# Autodesk Inventor assembly: Assembly2
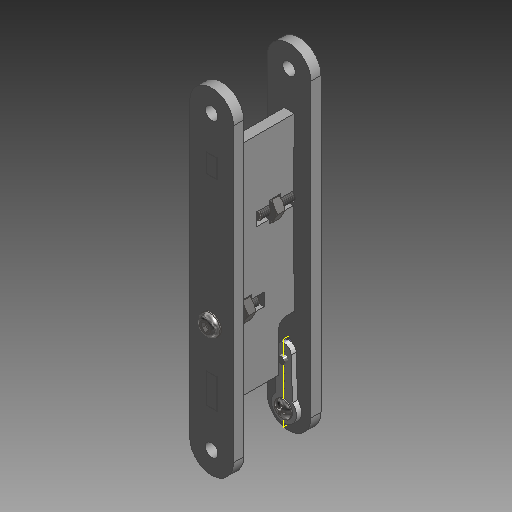
[picture p0: Inventor's stored thumbnail of the model, 512x512]
Saved by Autodesk Inventor 2019.2 (Build 232265000, 265)
## iProperties
Part Number: Assembly2
Document SubType Name: Assembly
Designer: richard.girt
Mass: 11.832 g
Surface Area: 93.4327 cm^2
Volume: 8.95603 cm^3
Density: 1.32112 g/cm^3
Author: richard.girt
## Documents named in this file (10)
- C:\Users\richard.girt\Desktop\2 Axis robotic arm\Assembly2.iam
- C:\Users\richard.girt\Desktop\2 Axis robotic arm\Part14.ipt
- C:\Users\richard.girt\Desktop\2 Axis robotic arm\Part5.ipt
- C:\Users\richard.girt\Desktop\2 Axis robotic arm\Part6.ipt
- C:\Users\richard.girt\Desktop\2 Axis robotic arm\SG90Horn1.ipt
- C:\Users\richard.girt\Desktop\2 Axis robotic arm\ANSI B18.6.5M - M2.5x0.45 x 4(38).ipt
- C:\Users\richard.girt\Desktop\2 Axis robotic arm\ANSI B18.6.5M - M2.5x0.45 x 8(38).ipt
- ANSI B18.6.5M - M2.5x0.45 x 8(38).ipt
- C:\Users\richard.girt\Desktop\2 Axis robotic arm\ANSI B 18.2.4.1 M - M3 x 0.5Style 1.ipt
- C:\Users\richard.girt\Desktop\2 Axis robotic arm\ANSI B18.3.4M - M3 x 0.5 x 12(1).ipt
## Components (10 placed, 8 different names)
1. Part14:1 — Flush:1, Flush:2, Flush:3, Flush:4, Mate:2
2. Part5:1 — Flush:1, Mate:1, Flush:3, Rigid:4, Rigid:6
3. Part6:1 — Flush:2, Mate:1, Flush:4, Mate:2, Rigid:1, Rigid:5, Rigid:7
4. SG90Horn1:1 — Rigid:1, Rigid:2, Rigid:3
5. ANSI B18.6.5M - M2.5x0.45 x 4(38):1 — Rigid:2
6. ANSI B18.6.5M - M2.5x0.45 x 8(38):1 — Rigid:3
7. ANSI B 18.2.4.1 M - M3 x 0.5Style 1:1 — Rigid:7
8. ANSI B18.3.4M - M3 x 0.5 x 12(1):1 — Rigid:4
9. ANSI B18.3.4M - M3 x 0.5 x 12(1):2 — Rigid:5
10. ANSI B 18.2.4.1 M - M3 x 0.5Style 1:2 — Rigid:6
## Relationships (13: WeldJoint 7, Flush 4, Mate 2)
- Flush:1: Part14:1 ↔ Part5:1
- Flush:2: Part14:1 ↔ Part6:1
- Mate:1: Part5:1 ↔ Part6:1
- Flush:3: Part14:1 ↔ Part5:1
- Flush:4: Part14:1 ↔ Part6:1
- Mate:2 (10 mm): Part14:1 ↔ Part6:1
- Rigid:1 [WeldJoint]: Part6:1 ↔ SG90Horn1:1
- Rigid:2 [WeldJoint]: SG90Horn1:1 ↔ ANSI B18.6.5M - M2.5x0.45 x 4(38):1
- Rigid:3 [WeldJoint] (-2.8 mm): SG90Horn1:1 ↔ ANSI B18.6.5M - M2.5x0.45 x 8(38):1
- Rigid:4 [WeldJoint]: Part5:1 ↔ ANSI B18.3.4M - M3 x 0.5 x 12(1):1
- Rigid:5 [WeldJoint]: Part6:1 ↔ ANSI B18.3.4M - M3 x 0.5 x 12(1):2
- Rigid:6 [WeldJoint] (-4 mm): Part5:1 ↔ ANSI B 18.2.4.1 M - M3 x 0.5Style 1:2
- Rigid:7 [WeldJoint] (-4 mm): Part6:1 ↔ ANSI B 18.2.4.1 M - M3 x 0.5Style 1:1
